# Autodesk Inventor assembly: DIC3D
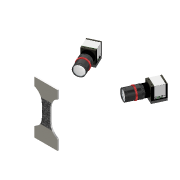
[picture p0: Inventor's stored thumbnail of the model, 180x180]
Saved by Autodesk Inventor 2021 (Build 250183000, 183)
## iProperties
Created: 2021-07-02
Part Number: DIC3D
Document SubType Name: Assembly
Designer: mcgheealex
Author: mcgheealex
## Documents named in this file (4)
- C:\Users\mcgheealex\Box\FranckLab_GUI\Icons\Figure creation\CadFiles\DIC3D.iam
- C:\Users\mcgheealex\Box\FranckLab_GUI\Icons\Figure creation\CadFiles\DCU223M-Solidworks.ipt
- C:\Users\mcgheealex\Box\FranckLab_GUI\Icons\Figure creation\CadFiles\Lens.ipt
- C:\Users\mcgheealex\Box\FranckLab_GUI\Icons\Figure creation\CadFiles\dogbone.ipt
## Components (5 placed, 3 different names)
1. DCU223M-Solidworks:1 — Mate:1, Mate:3
2. Lens:1 — Mate:1, Mate:3
3. dogbone:1
4. DCU223M-Solidworks:2
5. Lens:2
## Relationships (4: Mate 4)
- Mate:1: DCU223M-Solidworks:1 ↔ Lens:1
- Mate:3 (2.159 mm): DCU223M-Solidworks:1 ↔ Lens:1
- [Mate]: DCU223M-Solidworks:2 ↔ Lens:2
- [Mate] (2.159 mm): DCU223M-Solidworks:2 ↔ Lens:2
## Named parameters: d3_d0 = 0 mm, d4_d2 = 2.159 mm
